# Autodesk Inventor assembly: gear_MIR
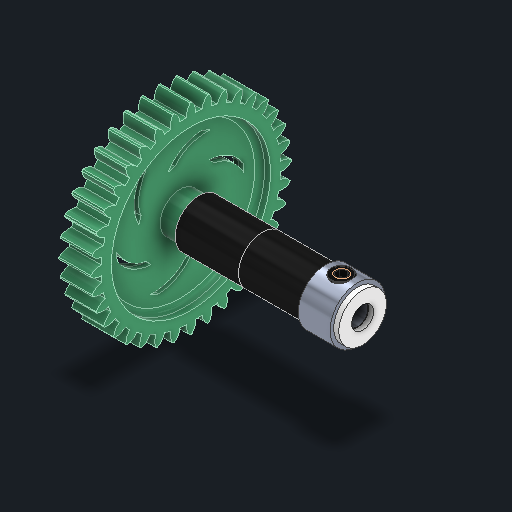
[picture p0: Inventor's stored thumbnail of the model, 512x512]
Saved by Autodesk Inventor 2024 (Build 280153000, 153)
## iProperties
Created: 2023-08-15
Part Number: gear_MIR
Document SubType Name: Assembly
Designer: avere
Author: avere
## Documents named in this file (9)
- D:\vex_robotics\hardware\cad\scrap_v0.1\chassis\mirrored_parts\gear_MIR.iam
- D:\vex_robotics\hardware\cad\scrap_v0.1\chassis\mirrored_parts\LS 36T Gear_MIR.ipt
- D:\vex_robotics\hardware\cad\VEX-CAD-Inventor-main\Motion\Spacers\Spacer Nylon .375 OD\NSpacer .375 OD x .500.ipt
- D:\vex_robotics\hardware\cad\VEX-CAD-Inventor-main\Motion\Spacers\Spacer Nylon .375 OD.ipt
- D:\vex_robotics\hardware\cad\scrap_v0.1\chassis\mirrored_parts\Shaft Collar Set Screw_MIR.ipt
- D:\vex_robotics\hardware\cad\VEX-CAD-Inventor-main\Motion\Spacers\Washer Teflon\TWasher .375 OD x .04000.ipt
- D:\vex_robotics\hardware\cad\VEX-CAD-Inventor-main\Motion\Spacers\Washer Teflon.ipt
- D:\vex_robotics\hardware\cad\VEX-CAD-Inventor-main\Motion\Spacers\Washer Steel\SWasher .375 OD x .015625.ipt
- D:\vex_robotics\hardware\cad\VEX-CAD-Inventor-main\Motion\Spacers\Washer Steel.ipt
## Components (6 placed, 5 different names)
1. LS 36T Gear_MIR:1 — Insert:1, Insert:4
2. NSpacer .375 OD x .500:1 — Insert:1, Insert:2
3. NSpacer .375 OD x .500:2 — Insert:2, Insert:3
4. Shaft Collar Set Screw_MIR:1 — Insert:3, Insert:5
5. TWasher .375 OD x .04000:1 — Insert:5
6. SWasher .375 OD x .015625:1 — Insert:4
## Relationships (5: Insert 5)
- Insert:1: LS 36T Gear_MIR:1 ↔ NSpacer .375 OD x .500:1
- Insert:2: NSpacer .375 OD x .500:1 ↔ NSpacer .375 OD x .500:2
- Insert:3: NSpacer .375 OD x .500:2 ↔ Shaft Collar Set Screw_MIR:1
- Insert:5: Shaft Collar Set Screw_MIR:1 ↔ TWasher .375 OD x .04000:1
- Insert:4: LS 36T Gear_MIR:1 ↔ SWasher .375 OD x .015625:1
